# Autodesk Inventor assembly: fc17_017
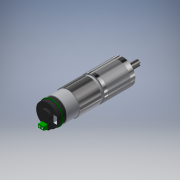
[picture p0: Inventor's stored thumbnail of the model, 180x180]
Saved by Autodesk Inventor 2017.1 (Build 211199000, 199)
## iProperties
Category: Motors
Company: Autodesk Inc.
Created: 2016-12-15
Part Number: fc17_017
Document SubType Name: Assembly
Designer: Autodesk Inc.
Catalog Web Link: http://www.andymark.com/product-p/am-2971.htm
Vendor: AndyMark Inc.
Author: Autodesk Inc.
Keywords: FIRSTChoice
## Documents named in this file (3)
- D:\FIRST\FIRST KOP 2017\FIRST FirstChoice 2017\fc17-017_GearMotorEncoder.iam
- D:\FIRST\FIRST KOP 2017\FIRST FirstChoice 2017\Parts\fc17-017_GearMotor.ipt
- D:\FIRST\FIRST KOP 2017\FIRST FirstChoice 2017\Parts\Hall Effect Encoder for PG Gearboxes.ipt
## Components (2 placed, 2 different names)
1. fc17-017_GearMotor:1 — Insert:1, Angle:1
2. Hall Effect Encoder for PG Gearboxes:1 — Insert:1, Angle:1
## Relationships (2: Insert 1, Angle 1)
- Insert:1: fc17-017_GearMotor:1 ↔ Hall Effect Encoder for PG Gearboxes:1
- Angle:1 (0 deg): fc17-017_GearMotor:1 ↔ Hall Effect Encoder for PG Gearboxes:1
